# Autodesk Inventor assembly: s-assy-shooter_unit
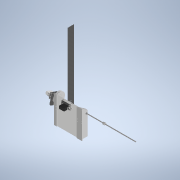
[picture p0: Inventor's stored thumbnail of the model, 180x180]
Saved by Autodesk Inventor 2022 (Build 260153000, 153)
## iProperties
Created: 2021-08-20
Part Number: s-assy-shooter_unit
Document SubType Name: Assembly
Designer: yuta0
Author: yuta0
## Documents named in this file (16)
- C:\Users\yuto6\Box\Public_Share\キャチロボバトルコンテスト2021\CAD\catchrobo_hardware\assy-shooter\s-assy-shooter_unit.iam
- C:\Users\yuto6\Box\Public_Share\キャチロボバトルコンテスト2021\CAD\catchrobo_hardware\assy-shooter\s_carbon_plate1.ipt
- C:\Users\yuto6\Box\Public_Share\キャチロボバトルコンテスト2021\CAD\catchrobo_hardware\assy-shooter\s_base2.ipt
- C:\Users\yuto6\Box\Public_Share\キャチロボバトルコンテスト2021\CAD\catchrobo_hardware\assy-shooter\s_base4.ipt
- C:\Users\yuto6\Box\Public_Share\キャチロボバトルコンテスト2021\CAD\catchrobo_hardware\assy-shooter\s-assy-guide_actuator.iam
- C:\Users\yuto6\Box\Public_Share\キャチロボバトルコンテスト2021\CAD\catchrobo_hardware\assy-shooter\MF126ZZ.ipt
- C:\Users\yuto6\Box\Public_Share\キャチロボバトルコンテスト2021\CAD\catchrobo_hardware\assy-shooter\CPRC16-6-6.iam
- C:\Users\yuto6\Box\Public_Share\キャチロボバトルコンテスト2021\CAD\catchrobo_hardware\assy-shooter\SCSTR6-8.iam
- C:\Users\yuto6\Box\Public_Share\キャチロボバトルコンテスト2021\CAD\catchrobo_hardware\assy-robot\CB4-10.ipt
- C:\Users\yuto6\Box\Public_Share\キャチロボバトルコンテスト2021\CAD\catchrobo_hardware\assy-shooter\s_carbon_plate5.ipt
- C:\Users\yuto6\Box\Public_Share\キャチロボバトルコンテスト2021\CAD\catchrobo_hardware\assy-shooter\s-assy-sorter.iam
- C:\Users\yuto6\Box\Public_Share\キャチロボバトルコンテスト2021\CAD\catchrobo_hardware\assy-shooter\PSFG6-350.ipt
- C:\Users\yuto6\Box\Public_Share\キャチロボバトルコンテスト2021\CAD\catchrobo_hardware\assy-shooter\PSFG6-270.ipt
- C:\Users\yuto6\Box\Public_Share\キャチロボバトルコンテスト2021\CAD\catchrobo_hardware\assy-shooter\s_carbon_plate6.ipt
- C:\Users\yuto6\Box\Public_Share\キャチロボバトルコンテスト2021\CAD\catchrobo_hardware\assy-shooter\s-assy-shooter_pulley.iam
- C:\Users\yuto6\Box\Public_Share\キャチロボバトルコンテスト2021\CAD\catchrobo_hardware\assy-robot\ARF-420E.ipt
## Components (23 placed, 15 different names)
1. s_base4:1 — メイト:20, メイト:21, フラッシュ:6, メイト:51, メイト:53, メイト:54, メイト:55, メイト:56, メイト:69, メイト:70, メイト:79, メイト:110, メイト:111, メイト:112, メイト:113, メイト:114, メイト:115, メイト:116
2. s-assy-guide_actuator:1 [sub-assembly] — メイト:51, メイト:69, メイト:70, フラッシュ:7, メイト:89, メイト:102, メイト:106, メイト:107, メイト:108, メイト:109
3. MF126ZZ:1 — メイト:53, メイト:54
4. MF126ZZ:2 — メイト:55, メイト:56
5. MF126ZZ:3 — メイト:58, メイト:59, メイト:83
6. MF126ZZ:4 — メイト:60, メイト:61, メイト:84
7. CPRC16-6-6:1 [sub-assembly] — メイト:65, メイト:84
8. s_carbon_plate5:1 — メイト:78, メイト:79, 角度:1, メイト:104, メイト:105
9. SCSTR6-8:1 [sub-assembly] — メイト:78, メイト:103, メイト:105
10. s_base2:1 — メイト:13, メイト:14, フラッシュ:5, メイト:58, メイト:59, メイト:60, メイト:61, メイト:65
11. s_carbon_plate1:1 — メイト:13, メイト:14, メイト:20, メイト:21, フラッシュ:5, フラッシュ:6, メイト:80, メイト:81, メイト:82, 角度:1
12. s-assy-sorter:1 [sub-assembly] — メイト:80, メイト:81, メイト:82
13. PSFG6-350:1 — メイト:83, フラッシュ:7, メイト:85, メイト:86, メイト:90, メイト:101, メイト:103, メイト:104
14. PSFG6-270:1 — メイト:85, メイト:86
15. s_carbon_plate6:1 — メイト:89, メイト:91, メイト:93, メイト:95, メイト:97, メイト:99, メイト:101, メイト:102, メイト:110, メイト:117
16. s-assy-shooter_pulley:1 [sub-assembly] — メイト:90, メイト:91
17. CB4-10:1 — メイト:93, メイト:107
18. CB4-10:2 — メイト:95, メイト:108
19. CB4-10:3 — メイト:97, メイト:109
20. CB4-10:4 — メイト:99, メイト:106
21. ARF-420E:2 — メイト:113, メイト:114
22. ARF-420E:3 — メイト:112, メイト:116
23. ARF-420E:4 — メイト:111, メイト:115, メイト:117
## Relationships (53: Mate 49, Flush 3, Angle 1)
- メイト:13 [Mate]: s_base2:1 ↔ s_carbon_plate1:1
- メイト:14 [Mate]: s_base2:1 ↔ s_carbon_plate1:1
- メイト:20 [Mate]: s_base4:1 ↔ s_carbon_plate1:1
- メイト:21 [Mate]: s_base4:1 ↔ s_carbon_plate1:1
- フラッシュ:5 [Flush]: s_base2:1 ↔ s_carbon_plate1:1
- フラッシュ:6 [Flush]: s_base4:1 ↔ s_carbon_plate1:1
- メイト:51 [Mate]: s_base4:1 ↔ s-assy-guide_actuator:1
- メイト:53 [Mate]: s_base4:1 ↔ MF126ZZ:1
- メイト:54 [Mate]: s_base4:1 ↔ MF126ZZ:1
- メイト:55 [Mate]: s_base4:1 ↔ MF126ZZ:2
- メイト:56 [Mate]: s_base4:1 ↔ MF126ZZ:2
- メイト:58 [Mate]: MF126ZZ:3 ↔ s_base2:1
- メイト:59 [Mate]: MF126ZZ:3 ↔ s_base2:1
- メイト:60 [Mate]: MF126ZZ:4 ↔ s_base2:1
- メイト:61 [Mate]: MF126ZZ:4 ↔ s_base2:1
- メイト:65 [Mate] (129.5 mm): CPRC16-6-6:1 ↔ s_base2:1
- メイト:69 [Mate]: s_base4:1 ↔ s-assy-guide_actuator:1
- メイト:70 [Mate]: s_base4:1 ↔ s-assy-guide_actuator:1
- メイト:78 [Mate]: s_carbon_plate5:1 ↔ SCSTR6-8:1
- メイト:79 [Mate] (87.5 mm): s_base4:1 ↔ s_carbon_plate5:1
- メイト:80 [Mate]: s_carbon_plate1:1 ↔ s-assy-sorter:1
- メイト:81 [Mate]: s_carbon_plate1:1 ↔ s-assy-sorter:1
- メイト:82 [Mate]: s_carbon_plate1:1 ↔ s-assy-sorter:1
- 角度:1 [Angle] (0 deg): s_carbon_plate5:1 ↔ s_carbon_plate1:1
- メイト:83 [Mate]: MF126ZZ:3 ↔ PSFG6-350:1
- フラッシュ:7 [Flush]: s-assy-guide_actuator:1 ↔ PSFG6-350:1
- メイト:84 [Mate]: MF126ZZ:4 ↔ CPRC16-6-6:1
- メイト:85 [Mate]: PSFG6-350:1 ↔ PSFG6-270:1
- メイト:86 [Mate]: PSFG6-350:1 ↔ PSFG6-270:1
- メイト:89 [Mate]: s-assy-guide_actuator:1 ↔ s_carbon_plate6:1
- メイト:90 [Mate]: PSFG6-350:1 ↔ s-assy-shooter_pulley:1
- メイト:91 [Mate] (5 mm): s_carbon_plate6:1 ↔ s-assy-shooter_pulley:1
- メイト:93 [Mate]: s_carbon_plate6:1 ↔ CB4-10:1
- メイト:95 [Mate]: s_carbon_plate6:1 ↔ CB4-10:2
- メイト:97 [Mate]: s_carbon_plate6:1 ↔ CB4-10:3
- メイト:99 [Mate]: s_carbon_plate6:1 ↔ CB4-10:4
- メイト:101 [Mate]: PSFG6-350:1 ↔ s_carbon_plate6:1
- メイト:102 [Mate]: s-assy-guide_actuator:1 ↔ s_carbon_plate6:1
- メイト:103 [Mate]: SCSTR6-8:1 ↔ PSFG6-350:1
- メイト:104 [Mate]: s_carbon_plate5:1 ↔ PSFG6-350:1
- メイト:105 [Mate]: s_carbon_plate5:1 ↔ SCSTR6-8:1
- メイト:106 [Mate]: s-assy-guide_actuator:1 ↔ CB4-10:4
- メイト:107 [Mate]: s-assy-guide_actuator:1 ↔ CB4-10:1
- メイト:108 [Mate]: s-assy-guide_actuator:1 ↔ CB4-10:2
- メイト:109 [Mate]: s-assy-guide_actuator:1 ↔ CB4-10:3
- メイト:110 [Mate]: s_base4:1 ↔ s_carbon_plate6:1
- メイト:111 [Mate]: s_base4:1 ↔ ARF-420E:4
- メイト:112 [Mate]: s_base4:1 ↔ ARF-420E:3
- メイト:113 [Mate]: s_base4:1 ↔ ARF-420E:2
- メイト:114 [Mate]: s_base4:1 ↔ ARF-420E:2
- メイト:115 [Mate]: s_base4:1 ↔ ARF-420E:4
- メイト:116 [Mate]: s_base4:1 ↔ ARF-420E:3
- メイト:117 [Mate]: s_carbon_plate6:1 ↔ ARF-420E:4
